# Autodesk Inventor assembly: Screen_Case
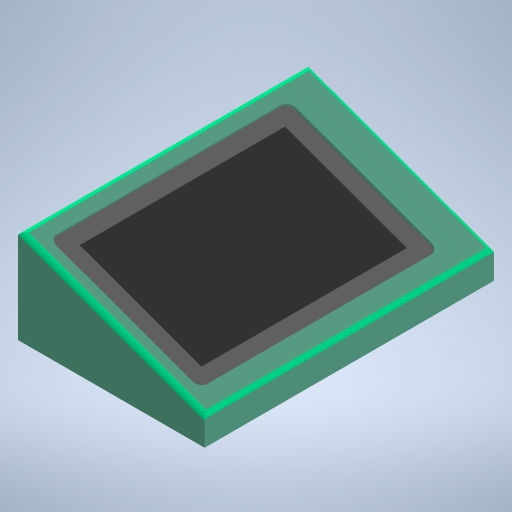
[picture p0: Inventor's stored thumbnail of the model, 512x512]
Saved by Autodesk Inventor 2024 (Build 280153000, 153)
## iProperties
Created: 2024-02-15
Part Number: Screen_Case
Document SubType Name: Assembly
Designer: fabiancastano
Author: fabiancastano
## Documents named in this file (4)
- C:\GitHub\PulseLaserPrj\CaseDesign\Case_parts\Screen_Case.iam
- C:\GitHub\PulseLaserPrj\CaseDesign\BaseFiles\LCD_10.1\LCD_10.1.iam
- C:\GitHub\PulseLaserPrj\CaseDesign\Case_parts\Screen_Support.ipt
- C:\GitHub\PulseLaserPrj\CaseDesign\Case_parts\screen_back_support_right.ipt
## Components (3 placed, 3 different names)
1. LCD_10.1:1 [sub-assembly] — Mate:1, Mate:2, Mate:3, Flush:1
2. Screen_Support:1 — Mate:1, Mate:2, Mate:3
3. screen_back_support_right:1 — Flush:1
## Relationships (4: Mate 3, Flush 1)
- Mate:1: LCD_10.1:1 ↔ Screen_Support:1
- Mate:2: LCD_10.1:1 ↔ Screen_Support:1
- Mate:3: LCD_10.1:1 ↔ Screen_Support:1
- Flush:1: LCD_10.1:1 ↔ screen_back_support_right:1
